# Autodesk Inventor assembly: suspension_one_side
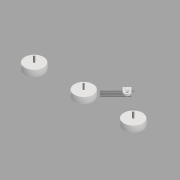
[picture p0: Inventor's stored thumbnail of the model, 180x180]
Saved by Autodesk Inventor 2021.3 (Build 253353000, 353)
## iProperties
Created: 2021-05-27
Part Number: suspension_one_side
Document SubType Name: Assembly
Designer: gisen
Author: gisen
## Documents named in this file (3)
- C:\Users\gisen\workspace\beetle_inventor_model\suspension\suspension_left.iam
- C:\Users\gisen\workspace\beetle_inventor_model\suspension\rocker.iam
- C:\Users\gisen\workspace\beetle_inventor_model\suspension\bogie.iam
## Components (2 placed, 2 different names)
1. rocker:1 [sub-assembly] — メイト:1, メイト:2
2. bogie:1 [sub-assembly] — メイト:1, メイト:2
## Relationships (2: Mate 2)
- メイト:1 [Mate]: rocker:1 ↔ bogie:1
- メイト:2 [Mate] (600 mm): rocker:1 ↔ bogie:1
